# Autodesk Inventor assembly: Reality
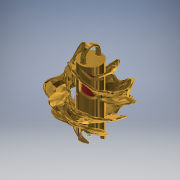
[picture p0: Inventor's stored thumbnail of the model, 180x180]
Saved by Autodesk Inventor 2019 (Build 230136000, 136)
## iProperties
Created: 2019-05-18
Part Number: Reality
Document SubType Name: Assembly
Designer: Jorian Brusind
Author: Jorian Brusind
## Documents named in this file (3)
- C:\Users\Jorian Brusind\Documents\GitHub\PersonalProjects\Inventor Projects\Infinity\Reality.iam
- C:\Users\Jorian Brusind\Documents\GitHub\PersonalProjects\Inventor Projects\Infinity\Waves.ipt
- C:\Users\Jorian Brusind\Documents\GitHub\PersonalProjects\Inventor Projects\Infinity\Red.ipt
## Components (2 placed, 2 different names)
1. Waves:1 — Mate:1, Mate:2
2. Red:1 — Mate:1, Mate:2
## Relationships (2: Mate 2)
- Mate:1: Waves:1 ↔ Red:1
- Mate:2: Waves:1 ↔ Red:1
